# Autodesk Inventor assembly: Wasabi
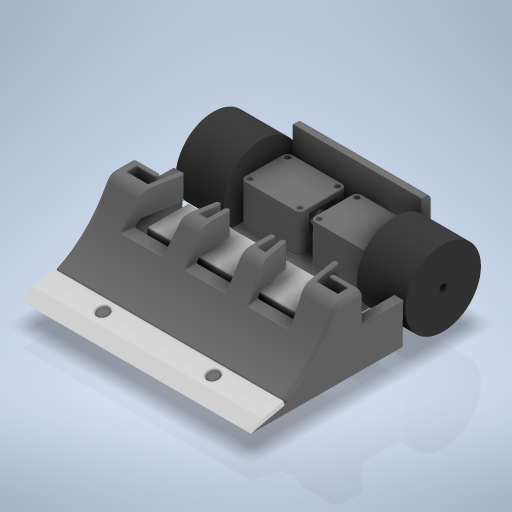
[picture p0: Inventor's stored thumbnail of the model, 512x512]
Saved by Autodesk Inventor 2024 (Build 280153000, 153)
## iProperties
Created: 2023-10-20
Part Number: Wasabi
Document SubType Name: Assembly
Designer: kdcao
Author: kdcao
## Documents named in this file (7)
- C:\Users\kdcao\Documents\wasabi2\Wasabi\Wasabi.iam
- C:\Users\kdcao\Documents\wasabi2\Wasabi\Body\Body.ipt
- C:\Users\kdcao\Documents\wasabi2\Wasabi\Parts\qtr-1a-reflectance-sensor.ipt
- C:\Users\kdcao\Documents\wasabi2\Wasabi\Parts\wheel.ipt
- C:\Users\kdcao\Documents\wasabi2\Wasabi\Parts\micro-metal-gearmotor-standard.ipt
- C:\Users\kdcao\Documents\wasabi2\Wasabi\Parts\Blade.ipt
- C:\Users\kdcao\Documents\wasabi2\Wasabi\Parts\BatteryV2.ipt
## Components (9 placed, 6 different names)
1. Body:1 — Tangent:2, Flush:5, Mate:5, Flush:6, Tangent:3, Tangent:4, Rigid:2, Rigid:3, Rigid:4, Mate:6, Mate:7, Mate:8, Mate:9
2. qtr-1a-reflectance-sensor:1 — Rigid:3
3. qtr-1a-reflectance-sensor:2 — Rigid:2
4. wheel:2 — Tangent:2, Flush:5, Cylindrical:1, Mate:4
5. micro-metal-gearmotor-standard:2 — Cylindrical:1, Mate:4, Mate:9
6. wheel:3 — Rotational:1, Flush:6, Tangent:3, Tangent:4
7. micro-metal-gearmotor-standard:3 — Mate:5, Rotational:1
8. Blade:1 — Rigid:4
9. BatteryV2:1 — Mate:6, Mate:7, Mate:8
## Relationships (16: Mate 6, Tangent 3, WeldJoint 3, Flush 2, CylindricalJoint 1, RevoluteJoint 1)
- Tangent:2 (1 mm): Body:1 ↔ wheel:2
- Flush:5: Body:1 ↔ wheel:2
- Cylindrical:1: wheel:2 ↔ micro-metal-gearmotor-standard:2
- Mate:4: wheel:2 ↔ micro-metal-gearmotor-standard:2
- Mate:5: Body:1 ↔ micro-metal-gearmotor-standard:3
- Rotational:1 [RevoluteJoint]: wheel:3 ↔ micro-metal-gearmotor-standard:3
- Flush:6: Body:1 ↔ wheel:3
- Tangent:3 (1 mm): Body:1 ↔ wheel:3
- Tangent:4 (1 mm): Body:1 ↔ wheel:3
- Rigid:2 [WeldJoint]: Body:1 ↔ qtr-1a-reflectance-sensor:2
- Rigid:3 [WeldJoint]: Body:1 ↔ qtr-1a-reflectance-sensor:1
- Rigid:4 [WeldJoint]: Body:1 ↔ Blade:1
- Mate:6: Body:1 ↔ BatteryV2:1
- Mate:7: Body:1 ↔ BatteryV2:1
- Mate:8: Body:1 ↔ BatteryV2:1
- Mate:9: Body:1 ↔ micro-metal-gearmotor-standard:2
